# Autodesk Inventor assembly: 足ユニット
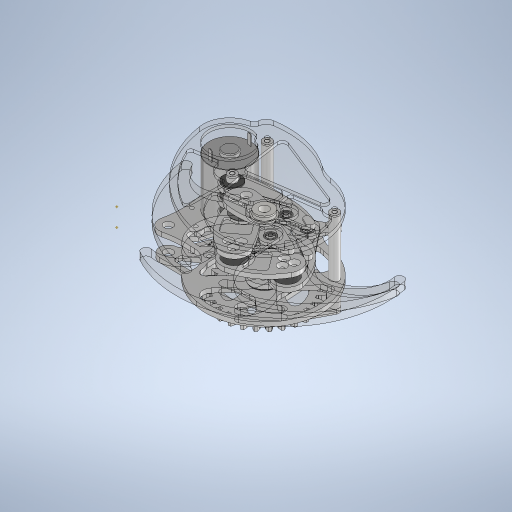
[picture p0: Inventor's stored thumbnail of the model, 512x512]
Saved by Autodesk Inventor 2023 (Build 270158000, 158)
## iProperties
Created: 2022-01-10
Part Number: 足ユニット
Document SubType Name: Assembly
Designer: acps
Author: acps
## Documents named in this file (19)
- C:\Users\acps\Documents\srdc\srdc_ksh\脚\足ユニット.iam
- C:\Users\acps\Documents\srdc\srdc_ksh\脚\足外フレーム.ipt
- C:\Users\acps\Documents\srdc\srdc_ksh\脚\足内フレーム.ipt
- C:\Users\acps\Documents\srdc\srdc_ksh\スペーサ\l40.ipt
- C:\Users\acps\Documents\srdc\srdc_ksh\カム\カム4.ipt
- C:\Users\acps\Documents\srdc\srdc_ksh\オイレス\w5f15-17n.ipt
- C:\Users\acps\Documents\srdc\srdc_ksh\モータ\M-RS-380.ipt
- C:\Users\acps\Documents\srdc\srdc_ksh\脚\ギア抑え.ipt
- C:\Users\acps\Documents\srdc\srdc_ksh\脚\モータマウント.ipt
- C:\Users\acps\Documents\srdc\srdc_ksh\ベアリング\Φ6-12a.ipt
- C:\Users\acps\Documents\srdc\srdc_ksh\脚\ギア\初段_多段ギア.iam
- C:\Users\acps\Documents\srdc\srdc_ksh\脚\ギア\ぴにょん.ipt
- C:\Users\acps\Documents\srdc\srdc_ksh\ベアリング\M-φ4φ8a.ipt
- C:\Users\acps\Documents\srdc\srdc_ksh\ピン\φ4ピン　L20.ipt
- C:\Users\acps\Documents\srdc\srdc_ksh\ベアリング\φ4φ8ベアリングa.ipt
- C:\Users\acps\Documents\srdc\srdc_ksh\スペーサ\l13.ipt
- C:\Users\acps\Documents\srdc\srdc_ksh\脚\ギア\最終段m2z28t4.ipt
- C:\Users\acps\Documents\srdc\srdc_ksh\脚\クランク.iam
- C:\Users\acps\Documents\srdc\srdc_ksh\脚\揺動節+ヘッケン.iam
## Components (25 placed, 18 different names)
1. l40:1 — Insert:22, Mate:47
2. l40:2 — Insert:21, Insert:27
3. l40:3 — Mate:30, Insert:23, Mate:49, Mate:51, Mate:53, Mate:55
4. カム4:1 — Insert:9, Mate:37, Mate:44, Mate:45, Insert:41, Insert:51
5. w5f15-17n:1 — Insert:9, Mate:29
6. M-RS-380:1 — Mate:27, Insert:31, Mate:38, Insert:32
7. ギア抑え:1 — Mate:36, Mate:37, Insert:36, Insert:38, Insert:53
8. Φ6-12a:1 — Insert:28, Mate:48, Insert:42
9. モータマウント:1 — Mate:35, Insert:30, Insert:31
10. 足内フレーム:1 — Mate:27, Mate:29, Insert:21, Insert:22, Mate:30, Insert:23, Mate:35, Insert:30, Mate:36, Mate:40, Insert:33, Insert:35, Insert:37, Insert:39, Insert:40
11. 足外フレーム:1 — Insert:27, Insert:28, Mate:47
12. ぴにょん:1 — Mate:38, Insert:32
13. M-φ4φ8a:1 — Mate:40, Insert:33, Mate:41, Mate:42
14. 初段_多段ギア:1 [sub-assembly] — Mate:41, Insert:53
15. φ4ピン　L20:1 — Mate:42, Insert:35, Mate:43
16. φ4φ8ベアリングa:1 — Mate:43, Insert:36
17. l13:1 — Insert:37, Insert:38
18. l13:2 — Insert:39
19. l13:3 — Insert:40
20. 最終段m2z28t4:1 — Mate:44, Mate:45, Insert:41
21. クランク:1 [sub-assembly] — Mate:48, Insert:42, Insert:51, Mate:50, Insert:52, Mate:52, Insert:54, Mate:54, Insert:55, Mate:56, Insert:56
22. 揺動節+ヘッケン:1 [sub-assembly] — Mate:51, Mate:52, Insert:54
23. 揺動節+ヘッケン:2 [sub-assembly] — Mate:53, Mate:54, Insert:55
24. 揺動節+ヘッケン:3 [sub-assembly] — Mate:55, Mate:56, Insert:56
25. 揺動節+ヘッケン:4 [sub-assembly] — Mate:49, Mate:50, Insert:52
## Relationships (47: Insert 24, Mate 23)
- Insert:9: カム4:1 ↔ w5f15-17n:1
- Mate:27: M-RS-380:1 ↔ 足内フレーム:1
- Mate:29: w5f15-17n:1 ↔ 足内フレーム:1
- Insert:21: l40:2 ↔ 足内フレーム:1
- Insert:22: l40:1 ↔ 足内フレーム:1
- Mate:30: l40:3 ↔ 足内フレーム:1
- Insert:23: l40:3 ↔ 足内フレーム:1
- Insert:27: l40:2 ↔ 足外フレーム:1
- Insert:28: Φ6-12a:1 ↔ 足外フレーム:1
- Mate:35: モータマウント:1 ↔ 足内フレーム:1
- Insert:30: モータマウント:1 ↔ 足内フレーム:1
- Insert:31: M-RS-380:1 ↔ モータマウント:1
- Mate:36: ギア抑え:1 ↔ 足内フレーム:1
- Mate:37: カム4:1 ↔ ギア抑え:1
- Mate:38: M-RS-380:1 ↔ ぴにょん:1
- Insert:32: M-RS-380:1 ↔ ぴにょん:1
- Mate:40: 足内フレーム:1 ↔ M-φ4φ8a:1
- Insert:33: 足内フレーム:1 ↔ M-φ4φ8a:1
- Mate:41: M-φ4φ8a:1 ↔ 初段_多段ギア:1
- Mate:42: M-φ4φ8a:1 ↔ φ4ピン　L20:1
- Insert:35: 足内フレーム:1 ↔ φ4ピン　L20:1
- Mate:43: φ4ピン　L20:1 ↔ φ4φ8ベアリングa:1
- Insert:36: ギア抑え:1 ↔ φ4φ8ベアリングa:1
- Insert:37: 足内フレーム:1 ↔ l13:1
- Insert:38: ギア抑え:1 ↔ l13:1
- Insert:39: 足内フレーム:1 ↔ l13:2
- Insert:40: 足内フレーム:1 ↔ l13:3
- Mate:44: カム4:1 ↔ 最終段m2z28t4:1
- Mate:45: カム4:1 ↔ 最終段m2z28t4:1
- Insert:41: カム4:1 ↔ 最終段m2z28t4:1
- Mate:47: l40:1 ↔ 足外フレーム:1
- Mate:48: Φ6-12a:1 ↔ クランク:1
- Insert:42: Φ6-12a:1 ↔ クランク:1
- Insert:51: カム4:1 ↔ クランク:1
- Mate:49: l40:3 ↔ 揺動節+ヘッケン:4
- Mate:50: クランク:1 ↔ 揺動節+ヘッケン:4
- Insert:52 (0.25 mm): クランク:1 ↔ 揺動節+ヘッケン:4
- Insert:53 (0.75 mm): ギア抑え:1 ↔ 初段_多段ギア:1
- Mate:51: l40:3 ↔ 揺動節+ヘッケン:1
- Mate:52: クランク:1 ↔ 揺動節+ヘッケン:1
- Insert:54 (0.25 mm): クランク:1 ↔ 揺動節+ヘッケン:1
- Mate:53: l40:3 ↔ 揺動節+ヘッケン:2
- Mate:54: クランク:1 ↔ 揺動節+ヘッケン:2
- Insert:55 (0.25 mm): クランク:1 ↔ 揺動節+ヘッケン:2
- Mate:55: l40:3 ↔ 揺動節+ヘッケン:3
- Mate:56: クランク:1 ↔ 揺動節+ヘッケン:3
- Insert:56 (0.25 mm): クランク:1 ↔ 揺動節+ヘッケン:3
